# Autodesk Inventor assembly: ASSEMBLY_Z_Axis_Belt_Tensioner
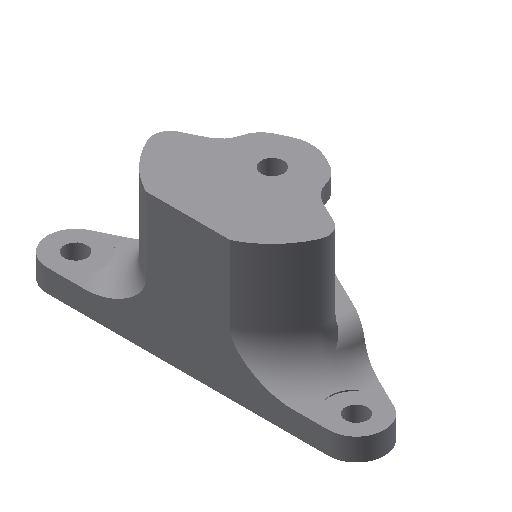
[picture p0: Inventor's stored thumbnail of the model, 512x512]
Saved by Autodesk Inventor 2026.1 (Build 301233000, 233)
## iProperties
Created: 2016-06-26
Part Number: ASSEMBLY_Z_Axis_Belt_Tensioner
Material: Ogólny
Document SubType Name: Assembly
Designer: Andrzej
Author: Andrzej
## Documents named in this file (3)
- C:\Users\Andrzej\OneDrive\_DRIVE_SYNCH_FILES\__ BYTECHLAB PROJECTS\MECH - FDM 3D Printer - RAPTOR-360\MCAD\1_REV1\ASSEMBLY_MAIN_REVA\ASSEMBLY_Z_Axis_Belt_Tensioner.iam
- C:\Users\Andrzej\OneDrive\_DRIVE_SYNCH_FILES\__ BYTECHLAB PROJECTS\MECH - FDM 3D Printer - RAPTOR-360\MCAD\1_REV1\ASSEMBLY_MAIN_REVA\3DP_ABS_Z_Axis_Belt_Tensioner.ipt
- C:\Users\Andrzej\OneDrive\_DRIVE_SYNCH_FILES\__ BYTECHLAB PROJECTS\MECH - FDM 3D Printer - RAPTOR-360\MCAD\1_REV1\__COTS_PARTS\COTS_GENERIC_604HZZ_Bearing.ipt
## Components (3 placed, 2 different names)
1. napinacz paska os Z:1 — Zestawiający:1, Zestawiający:3, Styczny:1
2. COTS_GENERIC_604HZZ_Bearing:1 — Zestawiający:2, Zestawiający:3, Styczny:1, Styczny:2
3. COTS_GENERIC_604HZZ_Bearing:2 — Zestawiający:1, Zestawiający:2, Styczny:2
## Relationships (5: Mate 3, Tangent 2)
- Zestawiający:1 [Mate] (1 mm): napinacz paska os Z:1 ↔ COTS_GENERIC_604HZZ_Bearing:2
- Zestawiający:2 [Mate]: COTS_GENERIC_604HZZ_Bearing:1 ↔ COTS_GENERIC_604HZZ_Bearing:2
- Zestawiający:3 [Mate] (2.25 mm): napinacz paska os Z:1 ↔ COTS_GENERIC_604HZZ_Bearing:1
- Styczny:1 [Tangent]: napinacz paska os Z:1 ↔ COTS_GENERIC_604HZZ_Bearing:1
- Styczny:2 [Tangent]: COTS_GENERIC_604HZZ_Bearing:1 ↔ COTS_GENERIC_604HZZ_Bearing:2
